# Autodesk Inventor assembly: Shadow_Game
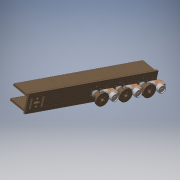
[picture p0: Inventor's stored thumbnail of the model, 180x180]
Saved by Autodesk Inventor 2016 (Build 200138000, 138)
## iProperties
Created: 2016-01-06
Part Number: Shadow_Game
Document SubType Name: Assembly
Designer: m2memari
Author: m2memari
## Documents named in this file (5)
- C:\MoDonGD\Jane\ShadowGame\ShadowGame\Shadow_Game.iam
- C:\MoDonGD\Jane\ShadowGame\ShadowGame\Motor_Bar.iam
- C:\MoDonGD\Jane\ShadowGame\ShadowGame\SPG30_Motor.ipt
- C:\MoDonGD\Jane\ShadowGame\ShadowGame\MotorCoupling.iam
- C:\MoDonGD\Jane\ShadowGame\ShadowGame\Bearing_Silicone.ipt
## Components (13 placed, 4 different names)
1. Motor_Bar:1 [sub-assembly] — Insert:1, Tangent:1, Flush:1, Mate:2, Mate:3, Mate:4, Mate:5, Mate:6, Mate:7, Flush:2, Flush:3, Mate:10, Mate:11, Mate:12, Mate:13, Mate:14, Mate:15, Mate:16, Mate:17, Mate:18, Mate:19, Mate:20, Mate:21
2. SPG30_Motor:1 — Insert:1, Tangent:1, Mate:1
3. MotorCoupling:1 [sub-assembly] — Mate:1, Flush:1
4. MotorCoupling:2 [sub-assembly] — Mate:9, Flush:3
5. SPG30_Motor:2 — Mate:3, Mate:5, Mate:7, Mate:9
6. SPG30_Motor:3 — Mate:2, Mate:4, Mate:6, Mate:8
7. MotorCoupling:3 [sub-assembly] — Mate:8, Flush:2
8. Bearing_Silicone:1 — Mate:10, Mate:11
9. Bearing_Silicone:2 — Mate:12, Mate:17
10. Bearing_Silicone:3 — Mate:13, Mate:18
11. Bearing_Silicone:4 — Mate:14, Mate:19
12. Bearing_Silicone:5 — Mate:15, Mate:20
13. Bearing_Silicone:6 — Mate:16, Mate:21
## Relationships (26: Mate 21, Flush 3, Insert 1, Tangent 1)
- Insert:1: Motor_Bar:1 ↔ SPG30_Motor:1
- Tangent:1: Motor_Bar:1 ↔ SPG30_Motor:1
- Mate:1: SPG30_Motor:1 ↔ MotorCoupling:1
- Flush:1: Motor_Bar:1 ↔ MotorCoupling:1
- Mate:2: Motor_Bar:1 ↔ SPG30_Motor:3
- Mate:3: Motor_Bar:1 ↔ SPG30_Motor:2
- Mate:4: Motor_Bar:1 ↔ SPG30_Motor:3
- Mate:5: Motor_Bar:1 ↔ SPG30_Motor:2
- Mate:6: Motor_Bar:1 ↔ SPG30_Motor:3
- Mate:7: Motor_Bar:1 ↔ SPG30_Motor:2
- Mate:8: SPG30_Motor:3 ↔ MotorCoupling:3
- Mate:9: MotorCoupling:2 ↔ SPG30_Motor:2
- Flush:2: Motor_Bar:1 ↔ MotorCoupling:3
- Flush:3: Motor_Bar:1 ↔ MotorCoupling:2
- Mate:10: Motor_Bar:1 ↔ Bearing_Silicone:1
- Mate:11: Motor_Bar:1 ↔ Bearing_Silicone:1
- Mate:12: Motor_Bar:1 ↔ Bearing_Silicone:2
- Mate:13: Motor_Bar:1 ↔ Bearing_Silicone:3
- Mate:14: Motor_Bar:1 ↔ Bearing_Silicone:4
- Mate:15: Motor_Bar:1 ↔ Bearing_Silicone:5
- Mate:16: Motor_Bar:1 ↔ Bearing_Silicone:6
- Mate:17: Motor_Bar:1 ↔ Bearing_Silicone:2
- Mate:18: Motor_Bar:1 ↔ Bearing_Silicone:3
- Mate:19: Motor_Bar:1 ↔ Bearing_Silicone:4
- Mate:20: Motor_Bar:1 ↔ Bearing_Silicone:5
- Mate:21: Motor_Bar:1 ↔ Bearing_Silicone:6
